# Autodesk Inventor assembly: Rodamiento mas arandela
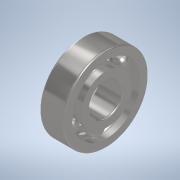
[picture p0: Inventor's stored thumbnail of the model, 180x180]
Saved by Autodesk Inventor 2021 (Build 250183000, 183)
## iProperties
Created: 2021-01-10
Part Number: Rodamiento mas arandela
Document SubType Name: Assembly
Designer: dieku
Author: dieku
## Documents named in this file (3)
- C:\Users\dieku\Documents\GitHub\tallerDibujoIngenieria\Ensambles\Rodamiento mas arandela.iam
- C:\Users\dieku\Documents\Inventor\Content Center Files\R2021\en-US\DIN 625 - T1\DIN 625 T1 - 6304 - 20 x 52 x 15.ipt
- C:\Users\dieku\Documents\GitHub\tallerDibujoIngenieria\Partes\UNE 18035.ipt
## Components (2 placed, 2 different names)
1. DIN 625 - T1 6304 - 20 x 52 x 15:1 — Mate:1
2. UNE 18035:1 — Mate:1
## Relationships (1: Mate 1)
- Mate:1: DIN 625 - T1 6304 - 20 x 52 x 15:1 ↔ UNE 18035:1
